# Autodesk Inventor assembly: Cage_connector_v01
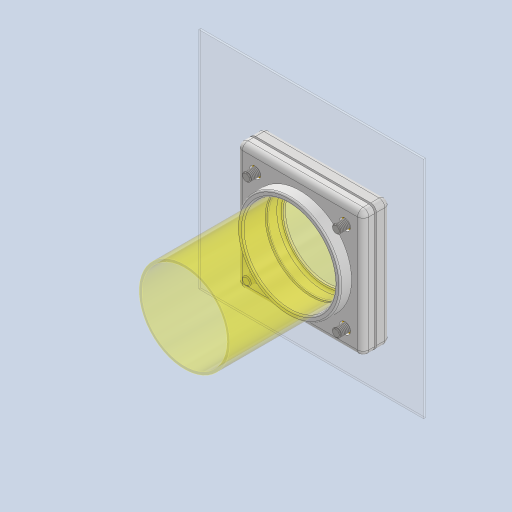
[picture p0: Inventor's stored thumbnail of the model, 512x512]
Saved by Autodesk Inventor 2024.4 (Build 284460000, 460)
## iProperties
Created: 2026-03-25
Part Number: Cage_connector_v01
Document SubType Name: Assembly
Designer: tooles01
Author: tooles01
## Documents named in this file (7)
- C:\Users\tooles01\NYU Langone Health Dropbox\Shannon Toole\Shannon_Dropbox\Mar lab\RFID\CAD\Cage_connector_v01.iam
- C:\Users\tooles01\NYU Langone Health Dropbox\Shannon Toole\Shannon_Dropbox\Mar lab\RFID\CAD\cage_inside_01.ipt
- C:\Users\tooles01\NYU Langone Health Dropbox\Shannon Toole\Shannon_Dropbox\Mar lab\RFID\CAD\cage_outside_01.ipt
- C:\Users\tooles01\NYU Langone Health Dropbox\Shannon Toole\Shannon_Dropbox\Mar lab\RFID\CAD\lib\cage_wall.ipt
- C:\Users\tooles01\NYU Langone Health Dropbox\Shannon Toole\Shannon_Dropbox\Mar lab\RFID\CAD\lib\M3 heat-set insert.ipt
- C:\Users\tooles01\Documents\Inventor\Content Center Files\R2024\en-US\AS 1420\AS 1420 - 1973 - M3 x 10.ipt
- C:\Users\tooles01\NYU Langone Health Dropbox\Shannon Toole\Shannon_Dropbox\Mar lab\RFID\CAD\lib\tube_5cm.ipt
## Components (12 placed, 6 different names)
1. cage_wall:1 — cage_outside to wall:1, cage_inside to wall:1
2. cage_inside_01:1 — cage_outside to wall:1, tube to cage_inside:1, screw to cage_outside:1, screw to cage_outside:2, screw to cage_outside:3, screw to cage_outside:4
3. cage_outside_01:1 — cage_inside to wall:1, heat-set to cage_outside:1, heat-set to cage_outside:2, heat-set to cage_outside:3, heat-set to cage_outside:4
4. tube_5cm:1 — tube to cage_inside:1
5. M3 heat-set insert:1 — heat-set to cage_outside:1
6. M3 heat-set insert:2 — heat-set to cage_outside:2
7. M3 heat-set insert:3 — heat-set to cage_outside:3
8. M3 heat-set insert:4 — heat-set to cage_outside:4
9. AS 1420 - Metric M3 x 10:1 — screw to cage_outside:1
10. AS 1420 - Metric M3 x 10:2 — screw to cage_outside:2
11. AS 1420 - Metric M3 x 10:3 — screw to cage_outside:3
12. AS 1420 - Metric M3 x 10:4 — screw to cage_outside:4
## Relationships (11: Insert 11)
- cage_outside to wall:1 [Insert]: cage_wall:1 ↔ cage_inside_01:1
- cage_inside to wall:1 [Insert]: cage_wall:1 ↔ cage_outside_01:1
- tube to cage_inside:1 [Insert]: cage_inside_01:1 ↔ tube_5cm:1
- heat-set to cage_outside:1 [Insert]: cage_outside_01:1 ↔ M3 heat-set insert:1
- heat-set to cage_outside:2 [Insert]: cage_outside_01:1 ↔ M3 heat-set insert:2
- heat-set to cage_outside:3 [Insert]: cage_outside_01:1 ↔ M3 heat-set insert:3
- heat-set to cage_outside:4 [Insert]: cage_outside_01:1 ↔ M3 heat-set insert:4
- screw to cage_outside:1 [Insert]: cage_inside_01:1 ↔ AS 1420 - Metric M3 x 10:1
- screw to cage_outside:2 [Insert]: cage_inside_01:1 ↔ AS 1420 - Metric M3 x 10:2
- screw to cage_outside:3 [Insert]: cage_inside_01:1 ↔ AS 1420 - Metric M3 x 10:3
- screw to cage_outside:4 [Insert]: cage_inside_01:1 ↔ AS 1420 - Metric M3 x 10:4
